# Autodesk Inventor assembly: 0304_練習2
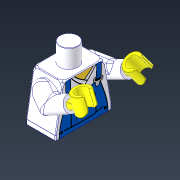
[picture p0: Inventor's stored thumbnail of the model, 180x180]
Saved by Autodesk Inventor 2022 (Build 260153000, 153)
## iProperties
Created: 2022-03-04
Part Number: 0304_練習2
Document SubType Name: Assembly
Designer: user
Author: user
## Documents named in this file (5)
- D:\pomelo\大一\下學期\機械設計製圖\PME1017_110033226\0304_練習2.iam
- D:\pomelo\大一\下學期\機械設計製圖\教材_LEGOmini_2022_20220218\X02598_LEGOmini_BackArmL_G.ipt
- D:\pomelo\大一\下學期\機械設計製圖\教材_LEGOmini_2022_20220218\X02598_LEGOmini_BackArmR_G.ipt
- D:\pomelo\大一\下學期\機械設計製圖\教材_LEGOmini_2022_20220218\X02598_LEGOmini_UpperBody.ipt
- D:\pomelo\大一\下學期\機械設計製圖\教材_LEGOmini_2022_20220218\X02598_LEGOmini_FrontArm_Y.ipt
## Components (5 placed, 4 different names)
1. X02598_LEGOmini_BackArmL_G:1 — 貼合:2, 貼合:3, 貼合:7, 貼合:8
2. X02598_LEGOmini_BackArmR_G:1 — 貼合:4, 貼合:5, 貼合:6, 貼合:9
3. X02598_LEGOmini_UpperBody:1 — 貼合:2, 貼合:3, 貼合:4, 貼合:5
4. X02598_LEGOmini_FrontArm_Y:1 — 貼合:6, 貼合:9
5. X02598_LEGOmini_FrontArm_Y:2 — 貼合:7, 貼合:8
## Relationships (8: Mate 8)
- 貼合:2 [Mate]: X02598_LEGOmini_BackArmL_G:1 ↔ X02598_LEGOmini_UpperBody:1
- 貼合:3 [Mate]: X02598_LEGOmini_BackArmL_G:1 ↔ X02598_LEGOmini_UpperBody:1
- 貼合:4 [Mate]: X02598_LEGOmini_BackArmR_G:1 ↔ X02598_LEGOmini_UpperBody:1
- 貼合:5 [Mate]: X02598_LEGOmini_BackArmR_G:1 ↔ X02598_LEGOmini_UpperBody:1
- 貼合:6 [Mate]: X02598_LEGOmini_BackArmR_G:1 ↔ X02598_LEGOmini_FrontArm_Y:1
- 貼合:7 [Mate]: X02598_LEGOmini_BackArmL_G:1 ↔ X02598_LEGOmini_FrontArm_Y:2
- 貼合:8 [Mate]: X02598_LEGOmini_BackArmL_G:1 ↔ X02598_LEGOmini_FrontArm_Y:2
- 貼合:9 [Mate]: X02598_LEGOmini_BackArmR_G:1 ↔ X02598_LEGOmini_FrontArm_Y:1
